# Autodesk Inventor assembly: SDA 63 50 Full_MIR
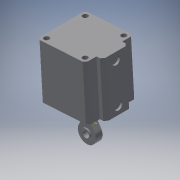
[picture p0: Inventor's stored thumbnail of the model, 180x180]
Saved by Autodesk Inventor 2019 (Build 230136000, 136)
## iProperties
Created: 2019-10-25
Part Number: SDA 63 50 Full_MIR
Document SubType Name: Assembly
Designer: Mark
Author: Mark
## Documents named in this file (4)
- C:\Users\Mark\Desktop\7738 Helion Engineering\7738-CAD-prep\Butterfly drive\SDA 63 50 Full_MIR.iam
- C:\Users\Mark\Desktop\7738 Helion Engineering\7738-CAD-prep\Butterfly drive\SDA 63 50_MIR.ipt
- C:\Users\Mark\Desktop\7738 Helion Engineering\7738-CAD-prep\Butterfly drive\SDA 63 50 Stroke Full_MIR.ipt
- C:\Users\Mark\Desktop\7738 Helion Engineering\7738-CAD-prep\Butterfly drive\SA10_MIR.iam
## Components (3 placed, 3 different names)
1. SDA 63 50_MIR:1 — Cylindrical:1
2. SDA 63 50 Stroke Full_MIR:1 — Insert:1, Cylindrical:1
3. SA10_MIR:1 [sub-assembly] — Insert:1
## Relationships (2: Insert 1, CylindricalJoint 1)
- Insert:1: SDA 63 50 Stroke Full_MIR:1 ↔ SA10_MIR:1
- Cylindrical:1: SDA 63 50_MIR:1 ↔ SDA 63 50 Stroke Full_MIR:1
